# Autodesk Inventor assembly: SimpleDesignV2 - 01
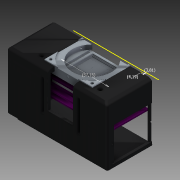
[picture p0: Inventor's stored thumbnail of the model, 180x180]
Saved by Autodesk Inventor 2015 (Build 190159000, 159)
## iProperties
Created: 2014-04-13
Part Number: SimpleDesignV2 - 01
Document SubType Name: Assembly
Designer: spichelh
Author: spichelh
## Documents named in this file (14)
- C:\Users\spichelh\Documents\GitHub\beta-hardware\Enclosure\SimpleDesign02\SimpleDesignV2 - 01.iam
- C:\Users\spichelh\Documents\GitHub\beta-hardware\Enclosure\SimpleDesign02\SFE-Host01.ipt
- C:\Users\spichelh\Documents\GitHub\beta-hardware\Enclosure\SimpleDesign02\SFE-ProcessingBoard01.ipt
- C:\Users\spichelh\Documents\GitHub\beta-hardware\Enclosure\SimpleDesign02\PCBModuleLeft02.ipt
- C:\Users\spichelh\Documents\GitHub\beta-hardware\Enclosure\SimpleDesign02\BetaBoard01.ipt
- C:\Users\spichelh\Documents\GitHub\beta-hardware\Enclosure\SimpleDesign02\Zynq_Z010_uZed_F_Prod.ipt
- C:\Users\spichelh\Documents\GitHub\beta-hardware\Enclosure\SimpleDesign02\PowerPCB01.ipt
- C:\Users\spichelh\Documents\GitHub\beta-hardware\Enclosure\SimpleDesign02\Samtec-PCIE-036-02-D-F-TH.ipt
- C:\Users\spichelh\Documents\GitHub\beta-hardware\Enclosure\SimpleDesign02\SensorCooler01.ipt
- C:\Users\spichelh\Documents\GitHub\beta-hardware\Enclosure\SimpleDesign02\CMV12000v1.ipt
- C:\Users\spichelh\Documents\GitHub\beta-hardware\Enclosure\SimpleDesign02\Sensormount_CMV12000-H.ipt
- C:\Users\spichelh\Documents\GitHub\beta-hardware\Enclosure\SimpleDesign02\threaded-rod01.ipt
- C:\Users\spichelh\Documents\GitHub\beta-hardware\Enclosure\SimpleDesign02\Simple3DPrintEnclosure01.ipt
- C:\Users\spichelh\Documents\GitHub\beta-hardware\Enclosure\SimpleDesign02\Simple3DPrintBackplate01.ipt
## Components (18 placed, 13 different names)
1. SFE-Host01:1 — Mate:73, Flush:48, Flush:49, Flush:125, Flush:126, Mate:163
2. SFE-ProcessingBoard01:1 — Mate:73, Flush:48, Flush:49, Flush:109, Mate:134, Flush:112, Mate:136, Flush:123, Flush:124, Mate:159
3. PCBModuleLeft02:1 — Flush:109, Mate:134, Flush:113, Flush:114
4. BetaBoard01:1 — Mate:135, Flush:110, Flush:111, Flush:112, Mate:136, Flush:113, Flush:114, Mate:137, Mate:138, Flush:115, Flush:116, Mate:142, Mate:143, Flush:117
5. Zynq_Z010_uZed_F_Prod:1 — Mate:131, Flush:107, Flush:108
6. PowerPCB01:1 — Mate:131, Flush:107, Flush:108, Mate:135, Flush:110, Flush:111
7. Samtec-PCIE-036-02-D-F-TH:1 — Mate:137, Mate:138, Flush:115, Flush:116
8. Samtec-PCIE-036-02-D-F-TH:2 — Mate:142, Mate:143, Flush:117
9. SensorCooler01:1
10. PCBModuleLeft02:2 — Flush:123, Flush:124, Mate:159
11. CMV12000v1:1 — Flush:125, Flush:126, Mate:163, Mate:164, Mate:165, Mate:166
12. Sensormount_CMV12000-H:1 — Mate:164, Mate:165, Mate:166, Mate:167, Flush:127, Mate:168, Mate:169, Mate:170, Mate:171, Flush:128, Flush:129, Mate:172, Flush:130, Flush:131, Mate:177, Mate:178
13. threaded-rod01:1 — Mate:168, Flush:128
14. threaded-rod01:2 — Mate:169, Flush:129
15. threaded-rod01:3 — Mate:170, Mate:171
16. threaded-rod01:4 — Mate:172, Flush:130
17. Simple3DPrintEnclosure01:1 — Flush:131, Mate:177, Mate:178, Mate:179, Mate:180, Mate:181
18. Simple3DPrintBackplate01:1 — Mate:179, Mate:180, Mate:181
## Relationships (47: Mate 25, Flush 22)
- Mate:73: SFE-Host01:1 ↔ SFE-ProcessingBoard01:1
- Flush:48: SFE-Host01:1 ↔ SFE-ProcessingBoard01:1
- Flush:49: SFE-Host01:1 ↔ SFE-ProcessingBoard01:1
- Mate:131 (7 mm): Zynq_Z010_uZed_F_Prod:1 ↔ PowerPCB01:1
- Flush:107: Zynq_Z010_uZed_F_Prod:1 ↔ PowerPCB01:1
- Flush:108: Zynq_Z010_uZed_F_Prod:1 ↔ PowerPCB01:1
- Flush:109: SFE-ProcessingBoard01:1 ↔ PCBModuleLeft02:1
- Mate:134 (1 mm): SFE-ProcessingBoard01:1 ↔ PCBModuleLeft02:1
- Mate:135 (5 mm): BetaBoard01:1 ↔ PowerPCB01:1
- Flush:110: BetaBoard01:1 ↔ PowerPCB01:1
- Flush:111: BetaBoard01:1 ↔ PowerPCB01:1
- Flush:112: SFE-ProcessingBoard01:1 ↔ BetaBoard01:1
- Mate:136: SFE-ProcessingBoard01:1 ↔ BetaBoard01:1
- Flush:113: PCBModuleLeft02:1 ↔ BetaBoard01:1
- Flush:114: PCBModuleLeft02:1 ↔ BetaBoard01:1
- Mate:137: BetaBoard01:1 ↔ Samtec-PCIE-036-02-D-F-TH:1
- Mate:138: BetaBoard01:1 ↔ Samtec-PCIE-036-02-D-F-TH:1
- Flush:115: BetaBoard01:1 ↔ Samtec-PCIE-036-02-D-F-TH:1
- Flush:116 (1.4908 mm): BetaBoard01:1 ↔ Samtec-PCIE-036-02-D-F-TH:1
- Mate:142: BetaBoard01:1 ↔ Samtec-PCIE-036-02-D-F-TH:2
- Mate:143: BetaBoard01:1 ↔ Samtec-PCIE-036-02-D-F-TH:2
- Flush:117 (2.0906 mm): BetaBoard01:1 ↔ Samtec-PCIE-036-02-D-F-TH:2
- Flush:123: SFE-ProcessingBoard01:1 ↔ PCBModuleLeft02:2
- Flush:124: SFE-ProcessingBoard01:1 ↔ PCBModuleLeft02:2
- Mate:159 (2 mm): SFE-ProcessingBoard01:1 ↔ PCBModuleLeft02:2
- Flush:125 (11.875 mm): SFE-Host01:1 ↔ CMV12000v1:1
- Flush:126 (5.175 mm): SFE-Host01:1 ↔ CMV12000v1:1
- Mate:163 (3 mm): SFE-Host01:1 ↔ CMV12000v1:1
- Mate:164: CMV12000v1:1 ↔ Sensormount_CMV12000-H:1
- Mate:165 (0.05 mm): CMV12000v1:1 ↔ Sensormount_CMV12000-H:1
- Mate:166: CMV12000v1:1 ↔ Sensormount_CMV12000-H:1
- Mate:167: Sensormount_CMV12000-H:1
- Flush:127: Sensormount_CMV12000-H:1
- Mate:168: Sensormount_CMV12000-H:1 ↔ threaded-rod01:1
- Mate:169: Sensormount_CMV12000-H:1 ↔ threaded-rod01:2
- Mate:170: Sensormount_CMV12000-H:1 ↔ threaded-rod01:3
- Mate:171: Sensormount_CMV12000-H:1 ↔ threaded-rod01:3
- Flush:128: Sensormount_CMV12000-H:1 ↔ threaded-rod01:1
- Flush:129: Sensormount_CMV12000-H:1 ↔ threaded-rod01:2
- Mate:172: Sensormount_CMV12000-H:1 ↔ threaded-rod01:4
- Flush:130: Sensormount_CMV12000-H:1 ↔ threaded-rod01:4
- Flush:131: Sensormount_CMV12000-H:1 ↔ Simple3DPrintEnclosure01:1
- Mate:177 (0.05 mm): Sensormount_CMV12000-H:1 ↔ Simple3DPrintEnclosure01:1
- Mate:178 (0.05 mm): Sensormount_CMV12000-H:1 ↔ Simple3DPrintEnclosure01:1
- Mate:179: Simple3DPrintEnclosure01:1 ↔ Simple3DPrintBackplate01:1
- Mate:180: Simple3DPrintEnclosure01:1 ↔ Simple3DPrintBackplate01:1
- Mate:181: Simple3DPrintEnclosure01:1 ↔ Simple3DPrintBackplate01:1
